# Autodesk Inventor assembly: Montagem
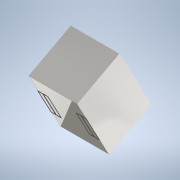
[picture p0: Inventor's stored thumbnail of the model, 180x180]
Saved by Autodesk Inventor 2022 (Build 260153000, 153)
## iProperties
Created: 2021-09-17
Part Number: Montagem
Document SubType Name: Assembly
Designer: rubia
Author: rubia
## Documents named in this file (4)
- C:\Users\rubia\Downloads\Montagem.iam
- C:\Users\rubia\Downloads\Grade.ipt
- C:\Users\rubia\Downloads\Caixa.ipt
- C:\Users\rubia\Downloads\PeçaFecha.ipt
## Components (5 placed, 3 different names)
1. Grade:1 — Coincidente:9, Coincidente:10, Coincidente:13
2. Grade:2 — Coincidente:11, Coincidente:12, Coincidente:14
3. Caixa:1 — Coincidente:3, Coincidente:4, Coincidente:5, Coincidente:6, Coincidente:7, Coincidente:8, Coincidente:9, Coincidente:10, Coincidente:11, Coincidente:12
4. PeçaFecha:1 — Coincidente:3, Coincidente:4, Coincidente:5
5. PeçaFecha:2 — Coincidente:6, Coincidente:7, Coincidente:8, Coincidente:13, Coincidente:14
## Relationships (12: Mate 12)
- Coincidente:3 [Mate]: Caixa:1 ↔ PeçaFecha:1
- Coincidente:4 [Mate]: Caixa:1 ↔ PeçaFecha:1
- Coincidente:5 [Mate]: Caixa:1 ↔ PeçaFecha:1
- Coincidente:6 [Mate]: Caixa:1 ↔ PeçaFecha:2
- Coincidente:7 [Mate]: Caixa:1 ↔ PeçaFecha:2
- Coincidente:8 [Mate]: Caixa:1 ↔ PeçaFecha:2
- Coincidente:9 [Mate]: Grade:1 ↔ Caixa:1
- Coincidente:10 [Mate]: Grade:1 ↔ Caixa:1
- Coincidente:11 [Mate]: Grade:2 ↔ Caixa:1
- Coincidente:12 [Mate]: Grade:2 ↔ Caixa:1
- Coincidente:13 [Mate] (100 mm): Grade:1 ↔ PeçaFecha:2
- Coincidente:14 [Mate] (100 mm): Grade:2 ↔ PeçaFecha:2
